# Autodesk Inventor assembly: servo assembly
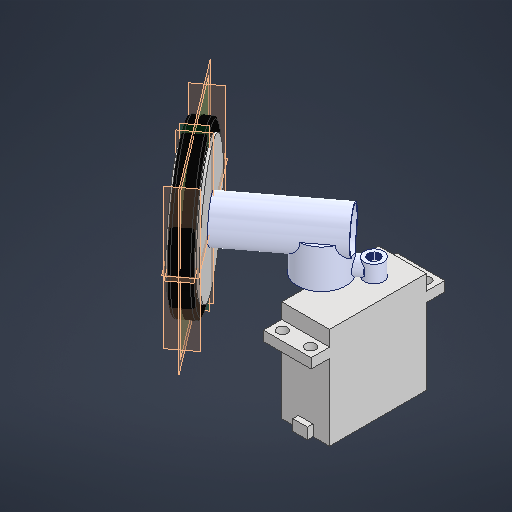
[picture p0: Inventor's stored thumbnail of the model, 512x512]
Saved by Autodesk Inventor 2026.2 (Build 302298000, 298)
## iProperties
Created: 2026-02-14
Part Number: servo assembly
Document SubType Name: Assembly
Designer: chigg
Author: chigg
## Documents named in this file (5)
- C:\Users\chigg\Robot_Spring_Semester\Robot_Model\servo assembly.iam
- C:\Users\chigg\Robot_Spring_Semester\Robot_Model\servo motor.ipt
- C:\Users\chigg\Robot_Spring_Semester\Robot_Model\Swivel_Part.ipt
- C:\Users\chigg\Robot_Spring_Semester\Robot_Model\14)_Wheel.ipt
- C:\Users\chigg\Robot_Spring_Semester\Robot_Model\13)_Rubber Wheel Cap.ipt
## Components (4 placed, 4 different names)
1. servo motor:1 — Rotational:1
2. Swivel_Part:1 — Insert:1, Rotational:1
3. 14)_Wheel:1 — Mate:2, Mate:3, Insert:1, Flush:1
4. 13)_Rubber Wheel Cap:1 — Mate:2, Mate:3, Flush:1
## Relationships (5: Mate 2, Insert 1, Flush 1, RevoluteJoint 1)
- Mate:2: 14)_Wheel:1 ↔ 13)_Rubber Wheel Cap:1
- Mate:3: 14)_Wheel:1 ↔ 13)_Rubber Wheel Cap:1
- Insert:1 (-10.0076 mm): Swivel_Part:1 ↔ 14)_Wheel:1
- Flush:1: 14)_Wheel:1 ↔ 13)_Rubber Wheel Cap:1
- Rotational:1 [RevoluteJoint] (4.318 mm): servo motor:1 ↔ Swivel_Part:1
